# Autodesk Inventor assembly: zlozenie
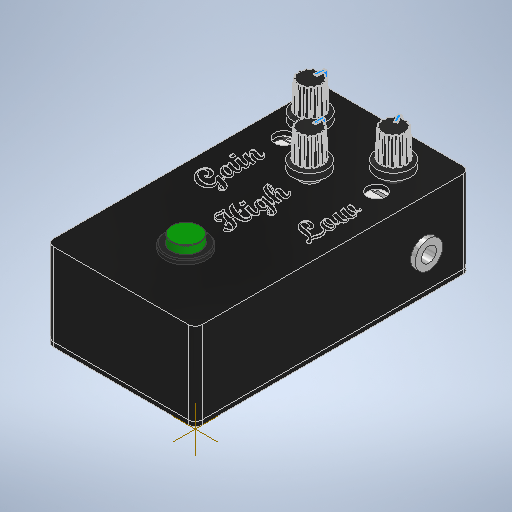
[picture p0: Inventor's stored thumbnail of the model, 512x512]
Saved by Autodesk Inventor 2025 (Build 290162000, 162)
## iProperties
Created: 2026-04-02
Part Number: zlozenie
Document SubType Name: Assembly
Designer: zzapa
Author: zzapa
## Documents named in this file (12)
- C:\Users\zzapa\Desktop\Projekty\elektronika\Efekt overdrive\zlozenie.iam
- C:\Users\zzapa\Desktop\Projekty\elektronika\Efekt overdrive\podstawa.ipt
- C:\Users\zzapa\Desktop\Projekty\elektronika\Efekt overdrive\obudowa.ipt
- C:\Users\zzapa\Documents\Inventor\Content Center Files\R2025\pl-PL\GB 809-88 B\Nut GB 809 B M2,5 x 6.ipt
- C:\Users\zzapa\Desktop\Projekty\elektronika\Efekt overdrive\PotentiometerB10K.ipt
- C:\Users\zzapa\Desktop\Projekty\elektronika\Efekt overdrive\knob.ipt
- C:\Users\zzapa\Desktop\Projekty\elektronika\Efekt overdrive\Jack_obudowa.ipt
- C:\Users\zzapa\Desktop\Projekty\elektronika\Efekt overdrive\Jack_srodek.ipt
- C:\Users\zzapa\Desktop\Projekty\elektronika\Efekt overdrive\plytka.ipt
- C:\Users\zzapa\Desktop\Projekty\elektronika\Efekt overdrive\9V_battery.ipt
- C:\Users\zzapa\Desktop\Projekty\elektronika\Efekt overdrive\Push_Button.ipt
- C:\Users\zzapa\Desktop\Projekty\elektronika\Efekt overdrive\9V_input.ipt
## Components (20 placed, 11 different names)
1. podstawa:1 — Zestawiające:1, Zestawiające:2, Zestawiające:3, Zestawiające:4, Zestawiające:9
2. obudowa:1 — Zestawiające:3, Zestawiające:4, Zestawiające:5, Równoległe:1, Zestawiające:6, Równoległe:2, Zestawiające:7, Równoległe:3, Zestawiające:8, Równoległe:4, Zestawiające:9, Zestawiające:10, Zestawiające:11, Zestawiające:12, Zestawiające:13, Zestawiające:14, Zestawiające:15, Zestawiające:23, Zestawiające:24, Zestawiające:25, Zestawiające:26, Zestawiające:27, Zestawiające:28, Zestawiające:29, Zestawiające:30, Zestawiające:31, Równoległe:5, Zestawiające:32, Zestawiające:33
3. Nut GB/T 809-1988 Type B M2,5x6:1 — Zestawiające:5, Równoległe:1, Kątowe:1
4. Nut GB/T 809-1988 Type B M2,5x6:2 — Zestawiające:6, Równoległe:2, Kątowe:2
5. Nut GB/T 809-1988 Type B M2,5x6:3 — Zestawiające:7, Równoległe:3, Kątowe:3
6. Nut GB/T 809-1988 Type B M2,5x6:4 — Zestawiające:8, Równoległe:4, Kątowe:4
7. PotentiometerB10K:1 — Zestawiające:10, Zestawiające:11, Kątowe:5, Zestawiające:18, Zestawiające:19
8. PotentiometerB10K:2 — Zestawiające:12, Zestawiające:15, Kątowe:6, Zestawiające:17, Zestawiające:20
9. PotentiometerB10K:3 — Zestawiające:13, Zestawiające:14, Kątowe:7, Zestawiające:16, Zestawiające:21
10. knob:1 — Zestawiające:17, Zestawiające:20
11. knob:2 — Zestawiające:16, Zestawiające:21
12. knob:3 — Zestawiające:18, Zestawiające:19
13. Jack_obudowa:1 — Zestawiające:22, Zestawiające:25, Kątowe:11
14. Jack_srodek:1 — Zestawiające:22, Zestawiające:23, Zestawiające:24, Kątowe:10
15. Jack_obudowa:2 — Zestawiające:26, Zestawiające:27, Kątowe:9
16. Jack_srodek:2 — Zestawiające:28, Zestawiające:29, Kątowe:8
17. plytka:1
18. 9V_battery:1
19. Push_Button:1 — Zestawiające:30, Zestawiające:31, Kątowe:12
20. 9V_input:1 — Równoległe:5, Zestawiające:32, Zestawiające:33
## Relationships (50: Mate 33, Angle 12, Flush 5)
- Zestawiające:1 [Mate]: podstawa:1
- Zestawiające:2 [Mate]: podstawa:1
- Zestawiające:3 [Mate]: podstawa:1 ↔ obudowa:1
- Zestawiające:4 [Mate]: podstawa:1 ↔ obudowa:1
- Zestawiające:5 [Mate]: obudowa:1 ↔ Nut GB/T 809-1988 Type B M2,5x6:1
- Równoległe:1 [Flush]: obudowa:1 ↔ Nut GB/T 809-1988 Type B M2,5x6:1
- Zestawiające:6 [Mate]: obudowa:1 ↔ Nut GB/T 809-1988 Type B M2,5x6:2
- Równoległe:2 [Flush]: obudowa:1 ↔ Nut GB/T 809-1988 Type B M2,5x6:2
- Zestawiające:7 [Mate]: obudowa:1 ↔ Nut GB/T 809-1988 Type B M2,5x6:3
- Równoległe:3 [Flush]: obudowa:1 ↔ Nut GB/T 809-1988 Type B M2,5x6:3
- Zestawiające:8 [Mate]: obudowa:1 ↔ Nut GB/T 809-1988 Type B M2,5x6:4
- Równoległe:4 [Flush]: obudowa:1 ↔ Nut GB/T 809-1988 Type B M2,5x6:4
- Kątowe:1 [Angle] (0 deg): Nut GB/T 809-1988 Type B M2,5x6:1
- Kątowe:2 [Angle] (0 deg): Nut GB/T 809-1988 Type B M2,5x6:2
- Kątowe:3 [Angle] (0 deg): Nut GB/T 809-1988 Type B M2,5x6:3
- Kątowe:4 [Angle] (0 deg): Nut GB/T 809-1988 Type B M2,5x6:4
- Zestawiające:9 [Mate]: podstawa:1 ↔ obudowa:1
- Zestawiające:10 [Mate]: obudowa:1 ↔ PotentiometerB10K:1
- Zestawiające:11 [Mate]: obudowa:1 ↔ PotentiometerB10K:1
- Zestawiające:12 [Mate]: obudowa:1 ↔ PotentiometerB10K:2
- Zestawiające:13 [Mate]: obudowa:1 ↔ PotentiometerB10K:3
- Zestawiające:14 [Mate]: obudowa:1 ↔ PotentiometerB10K:3
- Zestawiające:15 [Mate]: obudowa:1 ↔ PotentiometerB10K:2
- Kątowe:5 [Angle] (0 deg): PotentiometerB10K:1
- Kątowe:6 [Angle] (0 deg): PotentiometerB10K:2
- Kątowe:7 [Angle] (0 deg): PotentiometerB10K:3
- Zestawiające:16 [Mate]: PotentiometerB10K:3 ↔ knob:2
- Zestawiające:17 [Mate]: PotentiometerB10K:2 ↔ knob:1
- Zestawiające:18 [Mate]: PotentiometerB10K:1 ↔ knob:3
- Zestawiające:19 [Mate]: PotentiometerB10K:1 ↔ knob:3
- Zestawiające:20 [Mate]: PotentiometerB10K:2 ↔ knob:1
- Zestawiające:21 [Mate]: PotentiometerB10K:3 ↔ knob:2
- Zestawiające:22 [Mate]: Jack_obudowa:1 ↔ Jack_srodek:1
- Zestawiające:23 [Mate]: obudowa:1 ↔ Jack_srodek:1
- Zestawiające:24 [Mate]: obudowa:1 ↔ Jack_srodek:1
- Zestawiające:25 [Mate]: obudowa:1 ↔ Jack_obudowa:1
- Zestawiające:26 [Mate]: obudowa:1 ↔ Jack_obudowa:2
- Zestawiające:27 [Mate]: obudowa:1 ↔ Jack_obudowa:2
- Zestawiające:28 [Mate]: obudowa:1 ↔ Jack_srodek:2
- Zestawiające:29 [Mate]: obudowa:1 ↔ Jack_srodek:2
- Kątowe:8 [Angle] (0 deg): Jack_srodek:2
- Kątowe:9 [Angle] (0 deg): Jack_obudowa:2
- Kątowe:10 [Angle] (0 deg): Jack_srodek:1
- Kątowe:11 [Angle] (0 deg): Jack_obudowa:1
- Zestawiające:30 [Mate]: obudowa:1 ↔ Push_Button:1
- Zestawiające:31 [Mate]: obudowa:1 ↔ Push_Button:1
- Kątowe:12 [Angle] (0 deg): Push_Button:1
- Równoległe:5 [Flush]: obudowa:1 ↔ 9V_input:1
- Zestawiające:32 [Mate]: obudowa:1 ↔ 9V_input:1
- Zestawiające:33 [Mate]: obudowa:1 ↔ 9V_input:1
